# Autodesk Inventor assembly: Assembly2
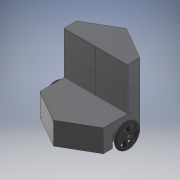
[picture p0: Inventor's stored thumbnail of the model, 180x180]
Saved by Autodesk Inventor 2017 (Build 210142000, 142)
## iProperties
Created: 2018-10-17
Part Number: Assembly2
Document SubType Name: Assembly
Designer: Administrator
Author: Administrator
## Documents named in this file (4)
- C:\Users\Dell\Documents\GitHub\tr2\Base\Base.iam
- C:\Users\Dell\Documents\GitHub\tr2\Wheel Assembly\Wheel Assembly.iam
- C:\Users\Dell\Documents\GitHub\tr2\Base\Base Cover Assembly.iam
- C:\Users\Dell\Documents\GitHub\tr2\Base\Base Chassis Assembly.iam
## Components (4 placed, 3 different names)
1. Wheel Assembly:1 [sub-assembly] — Mate:103
2. Wheel Assembly:2 [sub-assembly] — Mate:103, Mate:104, Mate:108
3. Base Cover Assembly:1 [sub-assembly]
4. Base Chassis Assembly:1 [sub-assembly] — Mate:104, Mate:105, Mate:106, Mate:107
## Relationships (46: Mate 36, Flush 10)
- [Mate]: Wheel Assembly:1 ↔ Base Chassis Assembly:1
- [Flush]: Wheel Assembly:1 ↔ Base Chassis Assembly:1
- [Mate]: Wheel Assembly:2 ↔ Base Chassis Assembly:1
- [Flush]: Wheel Assembly:2 ↔ Base Chassis Assembly:1
- [Mate]: Base Cover Assembly:1 ↔ Base Chassis Assembly:1
- [Flush]: Base Cover Assembly:1 ↔ Base Chassis Assembly:1
- [Mate]: Base Cover Assembly:1 ↔ Base Chassis Assembly:1
- [Mate]: Base Cover Assembly:1 ↔ Base Chassis Assembly:1
- [Flush]: Base Cover Assembly:1 ↔ Base Chassis Assembly:1
- [Flush]: Base Cover Assembly:1 ↔ Base Chassis Assembly:1
- [Mate]: Base Cover Assembly:1 ↔ Base Chassis Assembly:1
- [Flush]: Base Cover Assembly:1 ↔ Base Chassis Assembly:1
- [Mate]: Base Cover Assembly:1 ↔ Base Chassis Assembly:1
- [Mate]: Base Cover Assembly:1 ↔ Base Chassis Assembly:1
- [Mate]: Base Cover Assembly:1 ↔ Base Chassis Assembly:1
- [Flush]: Base Cover Assembly:1 ↔ Base Chassis Assembly:1
- [Mate]: Base Cover Assembly:1 ↔ Base Chassis Assembly:1
- [Flush]: Base Cover Assembly:1 ↔ Base Chassis Assembly:1
- [Mate]: Base Cover Assembly:1 ↔ Base Chassis Assembly:1
- [Flush]: Base Cover Assembly:1 ↔ Base Chassis Assembly:1
- [Mate]: Base Cover Assembly:1 ↔ Base Chassis Assembly:1
- [Flush]: Base Cover Assembly:1 ↔ Base Chassis Assembly:1
- [Mate]: Base Cover Assembly:1 ↔ Base Chassis Assembly:1
- [Mate]: Base Cover Assembly:1 ↔ Base Chassis Assembly:1
- [Mate]: Base Cover Assembly:1 ↔ Base Chassis Assembly:1
- [Mate]: Base Cover Assembly:1 ↔ Base Chassis Assembly:1
- [Mate]: Base Cover Assembly:1 ↔ Base Chassis Assembly:1
- [Mate]: Base Cover Assembly:1 ↔ Base Chassis Assembly:1
- [Mate]: Base Cover Assembly:1 ↔ Base Chassis Assembly:1
- [Mate]: Base Cover Assembly:1 ↔ Base Chassis Assembly:1
- [Mate]: Base Cover Assembly:1 ↔ Base Chassis Assembly:1
- [Mate]: Base Cover Assembly:1 ↔ Base Chassis Assembly:1
- [Mate]: Base Cover Assembly:1 ↔ Base Chassis Assembly:1
- [Mate]: Base Cover Assembly:1 ↔ Base Chassis Assembly:1
- [Mate]: Base Cover Assembly:1 ↔ Base Chassis Assembly:1
- [Mate]: Base Cover Assembly:1 ↔ Base Chassis Assembly:1
- [Mate]: Base Cover Assembly:1 ↔ Base Chassis Assembly:1
- [Mate]: Base Cover Assembly:1 ↔ Base Chassis Assembly:1
- [Mate]: Base Cover Assembly:1 ↔ Base Chassis Assembly:1
- [Mate]: Base Cover Assembly:1 ↔ Base Chassis Assembly:1
- Mate:103: Wheel Assembly:1 ↔ Wheel Assembly:2
- Mate:104 (131.025 mm): Wheel Assembly:2 ↔ Base Chassis Assembly:1
- Mate:105 (36.1 mm): Base Chassis Assembly:1
- Mate:106: Base Chassis Assembly:1
- Mate:107: Base Chassis Assembly:1
- Mate:108: Wheel Assembly:2
